# Autodesk Inventor assembly: Assey_Course_C_v1
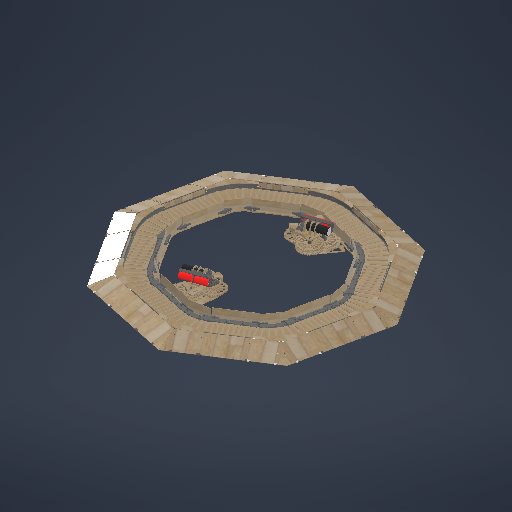
[picture p0: Inventor's stored thumbnail of the model, 512x512]
Saved by Autodesk Inventor 2026.3 (Build 303398000, 398)
## iProperties
Created: 2026-08-08
Part Number: Assey_Course_C_v1
Document SubType Name: Assembly
Designer: takuya
Author: takuya
## Documents named in this file (4)
- D:\model\D2_Conveyor_2026\Assey_Course_C.iam
- D:\model\D2_Conveyor_2026\power_module\Assy_power_module.iam
- D:\model\D2_Conveyor_2026\Assely_Curve_Liner.iam
- D:\model\D2_Conveyor_2026\curve_module\Assy_curve_module.iam
## Components (11 placed, 3 different names)
1. Assy_power_module:2 [sub-assembly] — メイト:36, 角度:2
2. Assy_power_module:3 [sub-assembly] — 角度:3, フラッシュ:16, メイト:76, メイト:77
3. Assy_power_module:4 [sub-assembly] — メイト:78, メイト:79
4. Assely_Curve_Liner:2 [sub-assembly] — メイト:65, フラッシュ:1, メイト:66, フラッシュ:14, フラッシュ:15, メイト:75
5. Assely_Curve_Liner:9 [sub-assembly] — フラッシュ:2, メイト:67, フラッシュ:3, フラッシュ:4, メイト:68, フラッシュ:5, メイト:78, メイト:79
6. Assy_curve_module:1 [sub-assembly] — メイト:65, フラッシュ:1, メイト:66, フラッシュ:2, メイト:67, フラッシュ:5
7. Assy_curve_module:2 [sub-assembly] — フラッシュ:3, フラッシュ:4, メイト:68
8. Assely_Curve_Liner:10 [sub-assembly] — メイト:73, フラッシュ:11, フラッシュ:13
9. Assely_Curve_Liner:11 [sub-assembly] — メイト:74, フラッシュ:10, フラッシュ:12, 角度:3, フラッシュ:16, メイト:76, メイト:77
10. Assy_curve_module:4 [sub-assembly] — フラッシュ:14, フラッシュ:15, メイト:75
11. Assy_curve_module:5 [sub-assembly] — メイト:73, メイト:74, フラッシュ:10, フラッシュ:11, フラッシュ:12, フラッシュ:13
## Relationships (33: Mate 17, Flush 14, Angle 2)
- メイト:36 [Mate]: Assy_power_module:2
- 角度:2 [Angle] (0 deg): Assy_power_module:2
- メイト:37 [Mate]
- メイト:62 [Mate]
- メイト:63 [Mate]
- メイト:64 [Mate]
- メイト:65 [Mate]: Assely_Curve_Liner:2 ↔ Assy_curve_module:1
- フラッシュ:1 [Flush]: Assely_Curve_Liner:2 ↔ Assy_curve_module:1
- メイト:66 [Mate]: Assely_Curve_Liner:2 ↔ Assy_curve_module:1
- フラッシュ:2 [Flush]: Assely_Curve_Liner:9 ↔ Assy_curve_module:1
- メイト:67 [Mate]: Assely_Curve_Liner:9 ↔ Assy_curve_module:1
- フラッシュ:3 [Flush]: Assely_Curve_Liner:9 ↔ Assy_curve_module:2
- フラッシュ:4 [Flush]: Assely_Curve_Liner:9 ↔ Assy_curve_module:2
- メイト:68 [Mate]: Assely_Curve_Liner:9 ↔ Assy_curve_module:2
- フラッシュ:5 [Flush]: Assely_Curve_Liner:9 ↔ Assy_curve_module:1
- [Flush]: Assely_Curve_Liner:11 ↔ Assy_curve_module:4
- [Flush]: Assely_Curve_Liner:11 ↔ Assy_curve_module:4
- [Mate]: Assely_Curve_Liner:11 ↔ Assy_curve_module:4
- メイト:73 [Mate]: Assely_Curve_Liner:10 ↔ Assy_curve_module:5
- メイト:74 [Mate]: Assely_Curve_Liner:11 ↔ Assy_curve_module:5
- フラッシュ:10 [Flush]: Assely_Curve_Liner:11 ↔ Assy_curve_module:5
- フラッシュ:11 [Flush]: Assely_Curve_Liner:10 ↔ Assy_curve_module:5
- フラッシュ:12 [Flush]: Assely_Curve_Liner:11 ↔ Assy_curve_module:5
- フラッシュ:13 [Flush]: Assely_Curve_Liner:10 ↔ Assy_curve_module:5
- フラッシュ:14 [Flush]: Assely_Curve_Liner:2 ↔ Assy_curve_module:4
- フラッシュ:15 [Flush]: Assely_Curve_Liner:2 ↔ Assy_curve_module:4
- メイト:75 [Mate]: Assely_Curve_Liner:2 ↔ Assy_curve_module:4
- 角度:3 [Angle] (0 deg): Assy_power_module:3 ↔ Assely_Curve_Liner:11
- フラッシュ:16 [Flush]: Assy_power_module:3 ↔ Assely_Curve_Liner:11
- メイト:76 [Mate]: Assy_power_module:3 ↔ Assely_Curve_Liner:11
- メイト:77 [Mate]: Assy_power_module:3 ↔ Assely_Curve_Liner:11
- メイト:78 [Mate]: Assy_power_module:4 ↔ Assely_Curve_Liner:9
- メイト:79 [Mate]: Assy_power_module:4 ↔ Assely_Curve_Liner:9
## Named parameters: d152_d150 = 0 mm, d159_d148 = 0 mm, d160_d149 = 0 mm
